# Autodesk Inventor assembly: BED ASSEMBLY
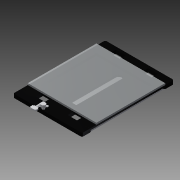
[picture p0: Inventor's stored thumbnail of the model, 180x180]
Saved by Autodesk Inventor 2013 (Build 170138000, 138)
## iProperties
Created: 2014-03-03
Part Number: BED ASSEMBLY
Document SubType Name: Assembly
Designer: employee
Author: employee
## Documents named in this file (7)
- C:\Users\employee\Desktop\CoreXZ\BED ASSEMBLY.iam
- C:\Users\employee\Desktop\CoreXZ\BED ROD MOUNT.ipt
- C:\Users\employee\Desktop\CoreXZ\M8X290 ROD.ipt
- C:\Users\employee\Desktop\CoreXZ\BED HOT BED INSET.ipt
- C:\Users\employee\Desktop\CoreXZ\GLASS.ipt
- C:\Users\employee\Desktop\CoreXZ\TUNING PEG.ipt
- C:\Users\employee\Desktop\CoreXZ\TUNING SPACER.ipt
## Components (7 placed, 6 different names)
1. BED ROD MOUNT:1 — Mate:1, Mate:2, Tangent:1, Tangent:2, Tangent:3, Tangent:4, Flush:1
2. M8X290 ROD:1 — Mate:2, Tangent:1, Tangent:2
3. M8X290 ROD:2 — Mate:1, Tangent:3, Tangent:4
4. BED HOT BED INSET:1 — Flush:1, Mate:3, Flush:2, Mate:4, Mate:5, Flush:3, Mate:6, Flush:4, Flush:5
5. GLASS:1 — Mate:3, Flush:2, Mate:4
6. TUNING PEG:1 — Mate:5, Flush:3, Mate:6
7. TUNING SPACER:1 — Flush:4, Flush:5
## Relationships (15: Mate 6, Flush 5, Tangent 4)
- Mate:1: BED ROD MOUNT:1 ↔ M8X290 ROD:2
- Mate:2: BED ROD MOUNT:1 ↔ M8X290 ROD:1
- Tangent:1: BED ROD MOUNT:1 ↔ M8X290 ROD:1
- Tangent:2: BED ROD MOUNT:1 ↔ M8X290 ROD:1
- Tangent:3: BED ROD MOUNT:1 ↔ M8X290 ROD:2
- Tangent:4: BED ROD MOUNT:1 ↔ M8X290 ROD:2
- Flush:1: BED ROD MOUNT:1 ↔ BED HOT BED INSET:1
- Mate:3: BED HOT BED INSET:1 ↔ GLASS:1
- Flush:2: BED HOT BED INSET:1 ↔ GLASS:1
- Mate:4 (-25.4 mm): BED HOT BED INSET:1 ↔ GLASS:1
- Mate:5 (6.477 mm): BED HOT BED INSET:1 ↔ TUNING PEG:1
- Flush:3: BED HOT BED INSET:1 ↔ TUNING PEG:1
- Mate:6 (-150 mm): BED HOT BED INSET:1 ↔ TUNING PEG:1
- Flush:4: BED HOT BED INSET:1 ↔ TUNING SPACER:1
- Flush:5: BED HOT BED INSET:1 ↔ TUNING SPACER:1
